# Autodesk Inventor assembly: Assembly small buttons
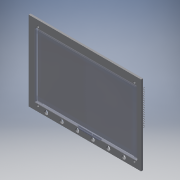
[picture p0: Inventor's stored thumbnail of the model, 180x180]
Saved by Autodesk Inventor 2019 (Build 230136000, 136)
## iProperties
Created: 2021-10-07
Part Number: Assembly small buttons
Document SubType Name: Assembly
Designer: maxwe
Author: maxwe
## Documents named in this file (3)
- D:\Makerplane_Efis\EFIS-Hardware-7-inch\New Enclosure\Assembly small buttons.iam
- D:\Makerplane_Efis\EFIS-Hardware-7-inch\New Enclosure\NHD-7.ipt
- D:\Makerplane_Efis\EFIS-Hardware-7-inch\New Enclosure\New Bezel.ipt
## Components (2 placed, 2 different names)
1. NHD-7:1 — Flush:1
2. New Bezel:1 — Flush:1
## Relationships (1: Flush 1)
- Flush:1: NHD-7:1 ↔ New Bezel:1
